# Autodesk Inventor assembly: TwoPartMQ-4Enclosure
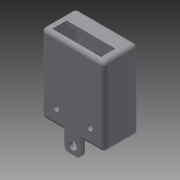
[picture p0: Inventor's stored thumbnail of the model, 180x180]
Saved by Autodesk Inventor 2014 SP1 (Build 180222100, 222)
## iProperties
Created: 2016-10-20
Part Number: TwoPartMQ-4Enclosure
Document SubType Name: Assembly
Designer: danielsikar
Author: danielsikar
## Documents named in this file (3)
- C:\Users\danielsikar\Documents\eagle\SLMS_Projects\MQ-4-IOT\enclosures\Assemblies\TwoPartMQ-4Enclosure.iam
- C:\Users\danielsikar\Documents\eagle\SLMS_Projects\MQ-4-IOT\enclosures\parts\bottom.ipt
- C:\Users\danielsikar\Documents\eagle\SLMS_Projects\MQ-4-IOT\enclosures\parts\top.ipt
## Components (2 placed, 2 different names)
1. bottom:1 — Flush:1, Flush:2, Mate:1
2. top:1 — Flush:1, Flush:2, Mate:1
## Relationships (3: Flush 2, Mate 1)
- Flush:1: bottom:1 ↔ top:1
- Flush:2: bottom:1 ↔ top:1
- Mate:1: bottom:1 ↔ top:1
